# Autodesk Inventor assembly: Сборка1
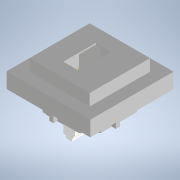
[picture p0: Inventor's stored thumbnail of the model, 180x180]
Saved by Autodesk Inventor 2021.2 (Build 252289000, 289)
## iProperties
Created: 2021-11-01
Part Number: Сборка1
Document SubType Name: Assembly
Designer: Kolan
Author: Kolan
## Documents named in this file (6)
- C:\_MCU\_Projects\SmartThings\SmartHeat\Inventor\Сборка1.iam
- C:\_MCU\_Projects\SmartThings\SmartHeat\Inventor\Плата печатная2.ipt
- C:\_MCU\_Projects\SmartThings\SmartHeat\Inventor\Низ.ipt
- C:\_MCU\_Projects\SmartThings\SmartHeat\Inventor\Середина.ipt
- C:\_MCU\_Projects\SmartThings\SmartHeat\Inventor\Середина 2.ipt
- C:\_MCU\_Projects\SmartThings\SmartHeat\Inventor\Верх.ipt
## Components (5 placed, 5 different names)
1. Плата печатная2:1 — Заподлицо:1
2. Низ:1 — Заподлицо:2, Заподлицо:3
3. Середина:1 — Заподлицо:3, Заподлицо:4
4. Середина 2:1 — Заподлицо:4, Заподлицо:5
5. Верх:1 — Заподлицо:5
## Relationships (5: Flush 5)
- Заподлицо:1 [Flush] (2 mm): Плата печатная2:1
- Заподлицо:2 [Flush]: Низ:1
- Заподлицо:3 [Flush]: Низ:1 ↔ Середина:1
- Заподлицо:4 [Flush]: Середина:1 ↔ Середина 2:1
- Заподлицо:5 [Flush]: Середина 2:1 ↔ Верх:1
